# Autodesk Inventor assembly: Assembly_box_2LED
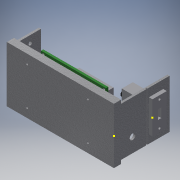
[picture p0: Inventor's stored thumbnail of the model, 180x180]
Saved by Autodesk Inventor 2018 (Build 220112000, 112)
## iProperties
Created: 2018-05-21
Part Number: Assembly_box_2LED
Document SubType Name: Assembly
Designer: David
Author: David
## Documents named in this file (5)
- C:\Users\David\Documents\optoelectronics\CAD\driver_box\Assembly_box_2LED.iam
- C:\Users\David\Documents\optoelectronics\CAD\driver_box\box.ipt
- C:\Users\David\Documents\optoelectronics\CAD\driver_box\PCB.ipt
- C:\Users\David\Documents\optoelectronics\CAD\usb-better-1.snapshot.4\USB_housing.ipt
- C:\Users\David\Documents\optoelectronics\CAD\usb-better-1.snapshot.4\usb head.ipt
## Components (4 placed, 4 different names)
1. box:1 — Mate:1, Mate:3, Mate:7, Mate:8, Mate:9, Mate:14
2. PCB:1 — Mate:1, Mate:3, Mate:7
3. USB_housing:1 — Mate:8, Mate:9, Mate:11, Mate:12, Mate:13, Mate:14
4. usb head:1 — Mate:11, Mate:12, Mate:13
## Relationships (9: Mate 9)
- Mate:1 (20 mm): box:1 ↔ PCB:1
- Mate:3: box:1 ↔ PCB:1
- Mate:7: box:1 ↔ PCB:1
- Mate:8: box:1 ↔ USB_housing:1
- Mate:9: box:1 ↔ USB_housing:1
- Mate:11: USB_housing:1 ↔ usb head:1
- Mate:12: USB_housing:1 ↔ usb head:1
- Mate:13 (0.475 mm): USB_housing:1 ↔ usb head:1
- Mate:14: box:1 ↔ USB_housing:1
